# Autodesk Inventor assembly: Assembly
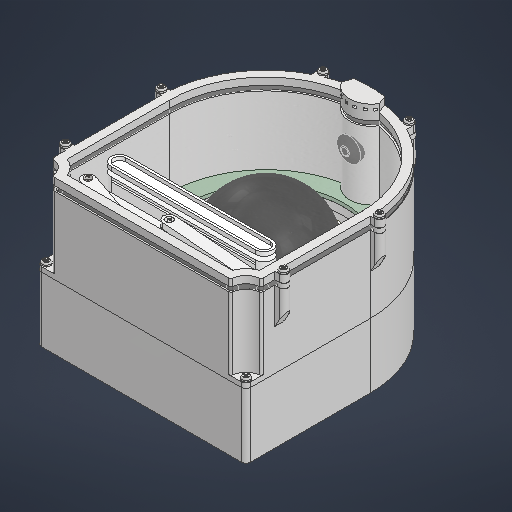
[picture p0: Inventor's stored thumbnail of the model, 512x512]
Saved by Autodesk Inventor 2026.2 (Build 302298000, 298)
## iProperties
Created: 2026-03-09
Part Number: Assembly
Document SubType Name: Assembly
Designer: Tathagata Sikdar
Author: Tathagata Sikdar
## Documents named in this file (17)
- D:\Productivity\Repos\early-lameness-detection\inventor_models\Assembly.iam
- D:\Productivity\Repos\early-lameness-detection\inventor_models\camera_base.ipt
- D:\Productivity\Repos\early-lameness-detection\inventor_models\wiper_arms.ipt
- D:\Productivity\Repos\early-lameness-detection\inventor_models\reservoir_cap.ipt
- D:\Productivity\Repos\early-lameness-detection\inventor_models\minipump\mini_pump.ipt
- D:\Productivity\Repos\early-lameness-detection\inventor_models\mcmaster_carr\7291N12_Wet-Environment Sealing Grommet\7291N12_Wet-Environment Sealing Grommet\7291N12_Wet-Environment Sealing Grommet.ipt
- D:\Productivity\Repos\early-lameness-detection\inventor_models\mcmaster_carr\99461A966_Phillips Rounded Head Thread-Forming Screws\99461A966_Phillips Rounded Head Thread-Forming Screws\99461A966_Phillips Rounde.ipt
- D:\Productivity\Repos\early-lameness-detection\inventor_models\mcmaster_carr\8785N395_Water- and Steam-Resistant EPDM O-Rings\8785N395_Water- and Steam-Resistant EPDM O-Rings\8785N395_Water- and Steam-Resistant.ipt
- D:\Productivity\Repos\early-lameness-detection\inventor_models\middle_gasket.ipt
- D:\Productivity\Repos\early-lameness-detection\inventor_models\upper_middle_gasket.ipt
- D:\Productivity\Repos\early-lameness-detection\inventor_models\Reolink Duo 3V\Reolink Duo 3V\Reolink Duo 3V.ipt
- D:\Productivity\Repos\early-lameness-detection\inventor_models\acrylic_clamp.ipt
- D:\Productivity\Repos\early-lameness-detection\inventor_models\top_gasket.ipt
- D:\Productivity\Repos\early-lameness-detection\inventor_models\acrylic_lens.ipt
- D:\Productivity\Repos\early-lameness-detection\inventor_models\spacer_4mm.ipt
- D:\Productivity\Repos\early-lameness-detection\inventor_models\wiper_assembly.iam
- D:\Productivity\Repos\early-lameness-detection\inventor_models\pcb.ipt
## Components (37 placed, 16 different names)
1. camera_base:1 — Flush:1, Flush:2, Flush:3, Flush:4, Flush:5, Flush:6, Flush:7, Mate:1, Angle:1, Mate:2, Mate:3, Insert:1, Insert:2, Insert:3, Insert:4, Mate:4, Mate:5, Mate:6, Flush:14, Insert:8
2. wiper_arms:1 — Flush:4
3. reservoir_cap:1 — Flush:5, Flush:6, Flush:7, Insert:5, Insert:6, Insert:7, Flush:15, Flush:16, Mate:7, Mate:8, Mate:9, Flush:18, Insert:15, Insert:16, Insert:17, Insert:18, Insert:19, Insert:20, Mate:11, Mate:12, Insert:21, Insert:22, Flush:19
4. mini_pump:1 — Mate:1, Angle:1, Mate:2, Mate:3
5. 7291N12_Wet-Environment Sealing Grommet:1 — Insert:1
6. 99461A966_Phillips Rounde:1 — Insert:5
7. 99461A966_Phillips Rounde:2 — Insert:3, Flush:10, Flush:11
8. 99461A966_Phillips Rounde:3 — Insert:4, Flush:8, Flush:9
9. 99461A966_Phillips Rounde:4 — Insert:2, Flush:12, Flush:13
10. 99461A966_Phillips Rounde:5 — Insert:6
11. 99461A966_Phillips Rounde:6 — Insert:7
12. 8785N395_Water- and Steam-Resistant:1 — Mate:4, Flush:8, Flush:9
13. 8785N395_Water- and Steam-Resistant:2 — Mate:5, Flush:10, Flush:11
14. 8785N395_Water- and Steam-Resistant:3 — Mate:6, Flush:12, Flush:13
15. middle_gasket:1 — Flush:14
16. upper_middle_gasket:1 — Flush:15
17. Reolink Duo 3V:1 — Insert:8
18. acrylic_clamp:1 — Flush:16, Flush:17, Insert:9, Insert:10, Insert:11, Insert:12, Insert:13, Insert:14
19. top_gasket:1 — Flush:17
20. top_gasket:2 — Mate:7, Mate:8, Mate:9
21. 99461A966_Phillips Rounde:7 — Insert:11
22. 99461A966_Phillips Rounde:8 — Insert:10
23. 99461A966_Phillips Rounde:9 — Insert:13
24. 99461A966_Phillips Rounde:10 — Insert:12
25. 99461A966_Phillips Rounde:11 — Insert:14
26. 99461A966_Phillips Rounde:12 — Insert:9
27. acrylic_lens:1 — Flush:18, Mate:10
28. spacer_4mm:1 — Insert:15
29. spacer_4mm:2 — Insert:20
30. spacer_4mm:3 — Insert:19
31. spacer_4mm:4 — Insert:16
32. spacer_4mm:5 — Insert:18
33. spacer_4mm:6 — Insert:17
34. wiper_assembly:1 [sub-assembly] — Mate:10, Mate:11, Mate:12
35. 7291N12_Wet-Environment Sealing Grommet:2 — Insert:21
36. 7291N12_Wet-Environment Sealing Grommet:3 — Insert:22
37. pcb:1 — Flush:19
## Relationships (54: Insert 22, Flush 19, Mate 12, Angle 1)
- Flush:1: camera_base:1
- Flush:2: camera_base:1
- Flush:3: camera_base:1
- Flush:4: camera_base:1 ↔ wiper_arms:1
- Flush:5: camera_base:1 ↔ reservoir_cap:1
- Flush:6: camera_base:1 ↔ reservoir_cap:1
- Flush:7: camera_base:1 ↔ reservoir_cap:1
- Mate:1: camera_base:1 ↔ mini_pump:1
- Angle:1 (0 deg): camera_base:1 ↔ mini_pump:1
- Mate:2: camera_base:1 ↔ mini_pump:1
- Mate:3 (20 mm): camera_base:1 ↔ mini_pump:1
- Insert:1: camera_base:1 ↔ 7291N12_Wet-Environment Sealing Grommet:1
- Insert:2: camera_base:1 ↔ 99461A966_Phillips Rounde:4
- Insert:3: camera_base:1 ↔ 99461A966_Phillips Rounde:2
- Insert:4: camera_base:1 ↔ 99461A966_Phillips Rounde:3
- Insert:5: reservoir_cap:1 ↔ 99461A966_Phillips Rounde:1
- Insert:6: reservoir_cap:1 ↔ 99461A966_Phillips Rounde:5
- Insert:7: reservoir_cap:1 ↔ 99461A966_Phillips Rounde:6
- Mate:4 (1 mm): camera_base:1 ↔ 8785N395_Water- and Steam-Resistant:1
- Flush:8: 99461A966_Phillips Rounde:3 ↔ 8785N395_Water- and Steam-Resistant:1
- Flush:9: 99461A966_Phillips Rounde:3 ↔ 8785N395_Water- and Steam-Resistant:1
- Mate:5 (1 mm): camera_base:1 ↔ 8785N395_Water- and Steam-Resistant:2
- Flush:10: 99461A966_Phillips Rounde:2 ↔ 8785N395_Water- and Steam-Resistant:2
- Flush:11: 99461A966_Phillips Rounde:2 ↔ 8785N395_Water- and Steam-Resistant:2
- Mate:6 (1 mm): camera_base:1 ↔ 8785N395_Water- and Steam-Resistant:3
- Flush:12: 99461A966_Phillips Rounde:4 ↔ 8785N395_Water- and Steam-Resistant:3
- Flush:13: 99461A966_Phillips Rounde:4 ↔ 8785N395_Water- and Steam-Resistant:3
- Flush:14 (2.5 mm): camera_base:1 ↔ middle_gasket:1
- Flush:15: reservoir_cap:1 ↔ upper_middle_gasket:1
- Insert:8: camera_base:1 ↔ Reolink Duo 3V:1
- Flush:16 (4 mm): reservoir_cap:1 ↔ acrylic_clamp:1
- Flush:17: acrylic_clamp:1 ↔ top_gasket:1
- Insert:9: acrylic_clamp:1 ↔ 99461A966_Phillips Rounde:12
- Insert:10: acrylic_clamp:1 ↔ 99461A966_Phillips Rounde:8
- Insert:11: acrylic_clamp:1 ↔ 99461A966_Phillips Rounde:7
- Insert:12: acrylic_clamp:1 ↔ 99461A966_Phillips Rounde:10
- Insert:13: acrylic_clamp:1 ↔ 99461A966_Phillips Rounde:9
- Insert:14: acrylic_clamp:1 ↔ 99461A966_Phillips Rounde:11
- Mate:7 (2.5 mm): reservoir_cap:1 ↔ top_gasket:2
- Mate:8 (2.5 mm): reservoir_cap:1 ↔ top_gasket:2
- Mate:9 (2.5 mm): reservoir_cap:1 ↔ top_gasket:2
- Flush:18: reservoir_cap:1 ↔ acrylic_lens:1
- Insert:15: reservoir_cap:1 ↔ spacer_4mm:1
- Insert:16: reservoir_cap:1 ↔ spacer_4mm:4
- Insert:17: reservoir_cap:1 ↔ spacer_4mm:6
- Insert:18: reservoir_cap:1 ↔ spacer_4mm:5
- Insert:19: reservoir_cap:1 ↔ spacer_4mm:3
- Insert:20: reservoir_cap:1 ↔ spacer_4mm:2
- Mate:10: acrylic_lens:1 ↔ wiper_assembly:1
- Mate:11: reservoir_cap:1 ↔ wiper_assembly:1
- Mate:12 (30 mm): reservoir_cap:1 ↔ wiper_assembly:1
- Insert:21: reservoir_cap:1 ↔ 7291N12_Wet-Environment Sealing Grommet:2
- Insert:22: reservoir_cap:1 ↔ 7291N12_Wet-Environment Sealing Grommet:3
- Flush:19: reservoir_cap:1 ↔ pcb:1
